# Autodesk Inventor assembly: 2020PiZeroCameraLightRingAssembly
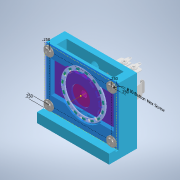
[picture p0: Inventor's stored thumbnail of the model, 180x180]
Saved by Autodesk Inventor 2020.2 (Build 242310000, 310)
## iProperties
Created: 2019-10-10
Part Number: 2020PiZeroCameraLightRingAssembly
Document SubType Name: Assembly
Designer: steele
Author: steele
## Documents named in this file (8)
- C:\git\CAD-Development\robSteele\2020PiZeroCameraLightRingMount\2020PiZeroCameraLightRingAssembly.iam
- C:\git\CAD-Development\robSteele\2020PiZeroCameraLightRingMount\2020PiZeroCameraLightRingMount.ipt
- C:\git\CAD-Development\robSteele\2020PiZeroCameraLightRingMount\RaspberryPiCameraCase.ipt
- C:\git\CAD-Development\robSteele\2020PiZeroCameraLightRingMount\fc18-097_RingLights.ipt
- C:\git\CAD-Development\robSteele\2020PiZeroCameraLightRingMount\2020LightRingCover.ipt
- C:\git\CAD-Development\robSteele\2020PiZeroCameraLightRingMount\2020PiZeroCameraLightRingAssembly\Design Accelerator\Bolted Connection1.iam
- C:\git\CAD-Development\robSteele\liftSpool\7712K620_BATTERY HOLDER.ipt
- C:\git\CAD-Development\robSteele\2020PiZeroCameraLightRingMount\2020PiZeroCameraLightRingAssembly\Design Accelerator\Bolted Connection2.iam
## Components (7 placed, 6 different names)
1. 2020PiZeroCameraLightRingMount:1 — Mate:1, Flush:1, Mate:2, Mate:3, Mate:4, Mate:5, Mate:6, Mate:9, Flush:2, Flush:3
2. RaspberryPiCameraCase:1 — Mate:1, Flush:1, Mate:2
3. fc18-097_RingLights:1 — Mate:3, Mate:4
4. 2020LightRingCover:1 — Mate:5, Mate:6, Mate:7, Mate:8
5. Bolted Connection:1 [sub-assembly] — Mate:7, Mate:8
6. 7712K620_BATTERY HOLDER:1 — Mate:9, Flush:2, Flush:3, Mate:10, Mate:11
7. Bolted Connection:2 [sub-assembly] — Mate:10, Mate:11
## Relationships (14: Mate 11, Flush 3)
- Mate:1: 2020PiZeroCameraLightRingMount:1 ↔ RaspberryPiCameraCase:1
- Flush:1: 2020PiZeroCameraLightRingMount:1 ↔ RaspberryPiCameraCase:1
- Mate:2: 2020PiZeroCameraLightRingMount:1 ↔ RaspberryPiCameraCase:1
- Mate:3: 2020PiZeroCameraLightRingMount:1 ↔ fc18-097_RingLights:1
- Mate:4: 2020PiZeroCameraLightRingMount:1 ↔ fc18-097_RingLights:1
- Mate:5: 2020PiZeroCameraLightRingMount:1 ↔ 2020LightRingCover:1
- Mate:6: 2020PiZeroCameraLightRingMount:1 ↔ 2020LightRingCover:1
- Mate:7: 2020LightRingCover:1 ↔ Bolted Connection:1
- Mate:8: 2020LightRingCover:1 ↔ Bolted Connection:1
- Mate:9: 2020PiZeroCameraLightRingMount:1 ↔ 7712K620_BATTERY HOLDER:1
- Flush:2 (-6.35 mm): 2020PiZeroCameraLightRingMount:1 ↔ 7712K620_BATTERY HOLDER:1
- Flush:3 (6.35 mm): 2020PiZeroCameraLightRingMount:1 ↔ 7712K620_BATTERY HOLDER:1
- Mate:10: 7712K620_BATTERY HOLDER:1 ↔ Bolted Connection:2
- Mate:11: 7712K620_BATTERY HOLDER:1 ↔ Bolted Connection:2
